# Autodesk Inventor assembly: ensembleFinal
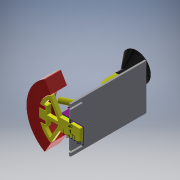
[picture p0: Inventor's stored thumbnail of the model, 180x180]
Saved by Autodesk Inventor 2019 (Build 230136000, 136)
## iProperties
Created: 2021-01-15
Part Number: ensembleFinal
Material: Générique
Document SubType Name: Assembly
Designer: tom.mousset
Author: tom.mousset
## Documents named in this file (6)
- D:\triSmarties\ensembleFinal.iam
- D:\triSmarties\pieceMere.ipt
- D:\triSmarties\bacRecupBonbon.ipt
- D:\triSmarties\EnsembleServoTobogan.iam
- D:\triSmarties\EnsembleV1.iam
- \\SRV-FICHIERS\tom.mousset$\Documents\planche.ipt
## Components (5 placed, 5 different names)
1. pieceMere:1 — Placage:1, Affleurement:1, Affleurement:2, Placage:2, Affleurement:3, Placage:7, Placage:8, Affleurement:4
2. bacRecupBonbon:1 — Placage:1, Affleurement:1, Affleurement:2, Placage:3
3. EnsembleServoTobogan:1 [sub-assembly] — Placage:2, Affleurement:3, Placage:3, Placage:4, Placage:5
4. EnsembleV1:1 [sub-assembly] — Placage:4, Placage:5, Angle:1
5. planche:1 — Placage:7, Placage:8, Affleurement:4, Angle:1
## Relationships (12: Mate 7, Flush 4, Angle 1)
- Placage:1 [Mate]: pieceMere:1 ↔ bacRecupBonbon:1
- Affleurement:1 [Flush]: pieceMere:1 ↔ bacRecupBonbon:1
- Affleurement:2 [Flush]: pieceMere:1 ↔ bacRecupBonbon:1
- Placage:2 [Mate] (15 mm): pieceMere:1 ↔ EnsembleServoTobogan:1
- Affleurement:3 [Flush] (11 mm): pieceMere:1 ↔ EnsembleServoTobogan:1
- Placage:3 [Mate]: bacRecupBonbon:1 ↔ EnsembleServoTobogan:1
- Placage:4 [Mate]: EnsembleServoTobogan:1 ↔ EnsembleV1:1
- Placage:5 [Mate] (20 mm): EnsembleServoTobogan:1 ↔ EnsembleV1:1
- Placage:7 [Mate]: pieceMere:1 ↔ planche:1
- Placage:8 [Mate]: pieceMere:1 ↔ planche:1
- Affleurement:4 [Flush] (30 mm): pieceMere:1 ↔ planche:1
- Angle:1 (0 deg): EnsembleV1:1 ↔ planche:1
